# Autodesk Inventor assembly: ASY TZS 0910 charging hatch
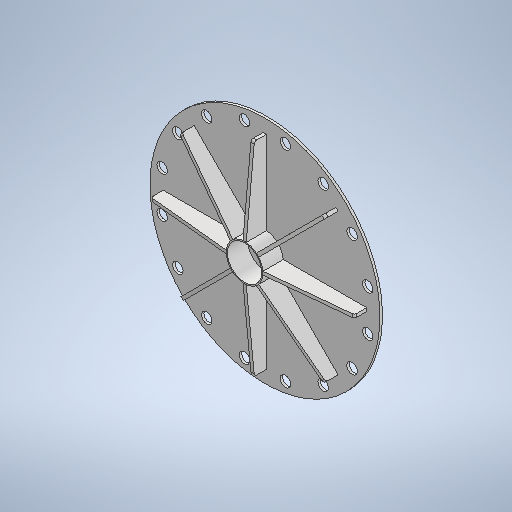
[picture p0: Inventor's stored thumbnail of the model, 512x512]
Saved by Autodesk Inventor 2025 (Build 290162010, 162A)
## iProperties
Created: 2025-04-22
Part Number: ASY TZS 0910 charging hatch
Document SubType Name: Assembly
Designer: user
Author: user
## Documents named in this file (4)
- C:\Users\pokla\Documents\Inventor\TZS-Tazovskiy\Filter D940\ASY TZS 0910 charging hatch.iam
- C:\Users\pokla\Documents\Inventor\TZS-Tazovskiy\Filter D940\TZS 0912 charging hatch 500 mm.ipt
- C:\Users\pokla\Documents\Inventor\TZS-Tazovskiy\Filter D940\TZS 0913 charging hatch reinf.ipt
- C:\Users\pokla\Documents\Inventor\TZS-Tazovskiy\Filter D940\TZS 0911 hatch tube 500mm.ipt
## Components (10 placed, 3 different names)
1. TZS 0912 charging hatch 500 mm.ipt:1 — Rigid:1, Flush:1
2. TZS 0911 hatch tube 500mm.ipt:1 — Rigid:1
3. TZS 0913 charging hatch reinf.ipt:1 — Mate:1, Flush:1, Mate:2, Mate:3
4. TZS 0913 charging hatch reinf.ipt:2
5. TZS 0913 charging hatch reinf.ipt:3
6. TZS 0913 charging hatch reinf.ipt:4
7. TZS 0913 charging hatch reinf.ipt:5
8. TZS 0913 charging hatch reinf.ipt:6
9. TZS 0913 charging hatch reinf.ipt:7
10. TZS 0913 charging hatch reinf.ipt:8
## Component patterns: (8 elements, first: TZS 0913 charging hatch reinf.ipt:1)
## Relationships (5: Mate 3, WeldJoint 1, Flush 1)
- Rigid:1 [WeldJoint]: TZS 0912 charging hatch 500 mm.ipt:1 ↔ TZS 0911 hatch tube 500mm.ipt:1
- Mate:1: TZS 0913 charging hatch reinf.ipt:1
- Flush:1: TZS 0912 charging hatch 500 mm.ipt:1 ↔ TZS 0913 charging hatch reinf.ipt:1
- Mate:2: TZS 0913 charging hatch reinf.ipt:1
- Mate:3: TZS 0913 charging hatch reinf.ipt:1
